# Autodesk Inventor assembly: X-Carriage_LM3011
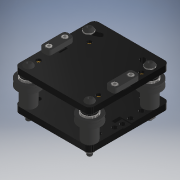
[picture p0: Inventor's stored thumbnail of the model, 180x180]
Saved by Autodesk Inventor 2020.2 (Build 242310000, 310)
## iProperties
Created: 2020-04-03
Part Number: X-Carriage_LM3011
Document SubType Name: Assembly
Designer: rah75
Author: rah75
## Documents named in this file (11)
- C:\Users\rah75\Documents\GitHub\LETU-Maker\CAD\Autodesk Inventor\Base_3001-5999\X-Carriage\Assemblies\X-Carriage_LM3011.iam
- C:\Users\rah75\Documents\GitHub\LETU-Maker\CAD\Autodesk Inventor\Base_3001-5999\X-Carriage\Fabricated_Parts\X-Carraige_Plate_LM3010.ipt
- C:\Users\rah75\Documents\GitHub\LETU-Maker\CAD\Autodesk Inventor\Base_3001-5999\X-Carriage\Printed_Parts\X-Carraige_Spacer_Long_LM3008.ipt
- C:\Users\rah75\Documents\GitHub\LETU-Maker\CAD\Autodesk Inventor\Base_3001-5999\X-Carriage\Printed_Parts\X-Carraige_Spacer_Short_LM3009.ipt
- C:\Users\rah75\Documents\GitHub\LETU-Maker\CAD\Autodesk Inventor\Base_3001-5999\X-Carriage\Printed_Parts\X-Carriage_Belt_Clamp_LM3007.ipt
- C:\Users\rah75\Documents\GitHub\LETU-Maker\CAD\Autodesk Inventor\Stock_Components_1001-2999\Power_Transmission\Bearings\V-Groove_Bearing_5mm_LM1041.ipt
- C:\Users\rah75\Documents\GitHub\LETU-Maker\CAD\Autodesk Inventor\Stock_Components_1001-2999\Fasteners\Nuts\heat_insert_m3_LM1017.ipt
- C:\Users\rah75\Documents\GitHub\LETU-Maker\CAD\Autodesk Inventor\Stock_Components_1001-2999\Fasteners\Screws\SHCS_m3x8_LM1008.ipt
- C:\Users\rah75\Documents\GitHub\LETU-Maker\CAD\Autodesk Inventor\Stock_Components_1001-2999\Fasteners\Washers_Spacers\washer_m5_LM1002.ipt
- C:\Users\rah75\Documents\GitHub\LETU-Maker\CAD\Autodesk Inventor\Stock_Components_1001-2999\Fasteners\Screws\BHHS_m5x50_LM1006.ipt
- C:\Users\rah75\Documents\GitHub\LETU-Maker\CAD\Autodesk Inventor\Stock_Components_1001-2999\Fasteners\Nuts\hex_nut_m5_LM1020.ipt
## Components (40 placed, 10 different names)
1. X-Carraige_Plate_LM3010:1 — Insert:8, Insert:9, Insert:10, Insert:11, Insert:14, Insert:15, Mate:1, Mate:2, Insert:16, Insert:17, Insert:18, Insert:19, Insert:20, Insert:21, Insert:22, Insert:23, Insert:30, Insert:31
2. X-Carraige_Plate_LM3010:2 — Insert:13, Insert:34, Insert:35, Insert:37, Insert:38
3. X-Carraige_Spacer_Long_LM3008:1 — Insert:12
4. X-Carraige_Spacer_Short_LM3009:1 — Insert:4, Insert:9
5. X-Carraige_Spacer_Long_LM3008:2 — Insert:7
6. X-Carraige_Spacer_Short_LM3009:2 — Insert:3, Insert:8
7. X-Carraige_Spacer_Long_LM3008:3 — Insert:5, Insert:13
8. X-Carraige_Spacer_Short_LM3009:3 — Insert:2, Insert:11
9. X-Carraige_Spacer_Long_LM3008:4 — Insert:6
10. X-Carraige_Spacer_Short_LM3009:4 — Insert:1, Insert:10
11. X-Carriage_Belt_Clamp_LM3007:1 — Insert:15, Mate:2, Insert:26, Insert:27
12. X-Carriage_Belt_Clamp_LM3007:2 — Insert:14, Mate:1, Insert:24, Insert:25
13. V-Groove_Bearing_5mm_LM1041:1 — Insert:4, Insert:7
14. V-Groove_Bearing_5mm_LM1041:2 — Insert:3, Insert:5
15. V-Groove_Bearing_5mm_LM1041:3 — Insert:2, Insert:12
16. V-Groove_Bearing_5mm_LM1041:4 — Insert:1, Insert:6
17. heat_insert_m3_LM1017:1 — Insert:18
18. heat_insert_m3_LM1017:2 — Insert:20
19. heat_insert_m3_LM1017:3 — Insert:17
20. heat_insert_m3_LM1017:4 — Insert:16
21. heat_insert_m3_LM1017:5 — Insert:22
22. heat_insert_m3_LM1017:6 — Insert:21
23. heat_insert_m3_LM1017:7 — Insert:23
24. heat_insert_m3_LM1017:8 — Insert:19
25. SHCS_m3x8_LM1008:1 — Insert:24
26. SHCS_m3x8_LM1008:2 — Insert:26
27. SHCS_m3x8_LM1008:3 — Insert:27
28. SHCS_m3x8_LM1008:4 — Insert:25
29. BHHS_m5x50_LM1006:1
30. BHHS_m5x50_LM1006:2
31. BHHS_m5x50_LM1006:3
32. BHHS_m5x50_LM1006:4
33. washer_m5_LM1002:1 — Insert:35, Insert:39
34. washer_m5_LM1002:2 — Insert:34, Insert:36
35. washer_m5_LM1002:3 — Insert:31
36. washer_m5_LM1002:4 — Insert:30
37. hex_nut_m5_LM1020:1 — Insert:39
38. hex_nut_m5_LM1020:2 — Insert:38
39. hex_nut_m5_LM1020:3 — Insert:37
40. hex_nut_m5_LM1020:4 — Insert:36
## Relationships (41: Insert 39, Mate 2)
- Insert:1: X-Carraige_Spacer_Short_LM3009:4 ↔ V-Groove_Bearing_5mm_LM1041:4
- Insert:2: X-Carraige_Spacer_Short_LM3009:3 ↔ V-Groove_Bearing_5mm_LM1041:3
- Insert:3: X-Carraige_Spacer_Short_LM3009:2 ↔ V-Groove_Bearing_5mm_LM1041:2
- Insert:4: X-Carraige_Spacer_Short_LM3009:1 ↔ V-Groove_Bearing_5mm_LM1041:1
- Insert:5: X-Carraige_Spacer_Long_LM3008:3 ↔ V-Groove_Bearing_5mm_LM1041:2
- Insert:6: X-Carraige_Spacer_Long_LM3008:4 ↔ V-Groove_Bearing_5mm_LM1041:4
- Insert:7: X-Carraige_Spacer_Long_LM3008:2 ↔ V-Groove_Bearing_5mm_LM1041:1
- Insert:8: X-Carraige_Plate_LM3010:1 ↔ X-Carraige_Spacer_Short_LM3009:2
- Insert:9: X-Carraige_Plate_LM3010:1 ↔ X-Carraige_Spacer_Short_LM3009:1
- Insert:10: X-Carraige_Plate_LM3010:1 ↔ X-Carraige_Spacer_Short_LM3009:4
- Insert:11: X-Carraige_Plate_LM3010:1 ↔ X-Carraige_Spacer_Short_LM3009:3
- Insert:12: X-Carraige_Spacer_Long_LM3008:1 ↔ V-Groove_Bearing_5mm_LM1041:3
- Insert:13: X-Carraige_Plate_LM3010:2 ↔ X-Carraige_Spacer_Long_LM3008:3
- Insert:14: X-Carraige_Plate_LM3010:1 ↔ X-Carriage_Belt_Clamp_LM3007:2
- Insert:15: X-Carraige_Plate_LM3010:1 ↔ X-Carriage_Belt_Clamp_LM3007:1
- Mate:1: X-Carraige_Plate_LM3010:1 ↔ X-Carriage_Belt_Clamp_LM3007:2
- Mate:2: X-Carraige_Plate_LM3010:1 ↔ X-Carriage_Belt_Clamp_LM3007:1
- Insert:16: X-Carraige_Plate_LM3010:1 ↔ heat_insert_m3_LM1017:4
- Insert:17: X-Carraige_Plate_LM3010:1 ↔ heat_insert_m3_LM1017:3
- Insert:18: X-Carraige_Plate_LM3010:1 ↔ heat_insert_m3_LM1017:1
- Insert:19: X-Carraige_Plate_LM3010:1 ↔ heat_insert_m3_LM1017:8
- Insert:20: X-Carraige_Plate_LM3010:1 ↔ heat_insert_m3_LM1017:2
- Insert:21: X-Carraige_Plate_LM3010:1 ↔ heat_insert_m3_LM1017:6
- Insert:22: X-Carraige_Plate_LM3010:1 ↔ heat_insert_m3_LM1017:5
- Insert:23: X-Carraige_Plate_LM3010:1 ↔ heat_insert_m3_LM1017:7
- Insert:24: X-Carriage_Belt_Clamp_LM3007:2 ↔ SHCS_m3x8_LM1008:1
- Insert:25: X-Carriage_Belt_Clamp_LM3007:2 ↔ SHCS_m3x8_LM1008:4
- Insert:26: X-Carriage_Belt_Clamp_LM3007:1 ↔ SHCS_m3x8_LM1008:2
- Insert:27: X-Carriage_Belt_Clamp_LM3007:1 ↔ SHCS_m3x8_LM1008:3
- [Insert]: BHHS_m5x50_LM1006:4 ↔ washer_m5_LM1002:3
- [Insert]: BHHS_m5x50_LM1006:3 ↔ washer_m5_LM1002:4
- Insert:30: X-Carraige_Plate_LM3010:1 ↔ washer_m5_LM1002:4
- Insert:31: X-Carraige_Plate_LM3010:1 ↔ washer_m5_LM1002:3
- [Insert]: X-Carraige_Plate_LM3010:1 ↔ BHHS_m5x50_LM1006:1
- [Insert]: X-Carraige_Plate_LM3010:1 ↔ BHHS_m5x50_LM1006:2
- Insert:34: X-Carraige_Plate_LM3010:2 ↔ washer_m5_LM1002:2
- Insert:35: X-Carraige_Plate_LM3010:2 ↔ washer_m5_LM1002:1
- Insert:36: washer_m5_LM1002:2 ↔ hex_nut_m5_LM1020:4
- Insert:37: X-Carraige_Plate_LM3010:2 ↔ hex_nut_m5_LM1020:3
- Insert:38: X-Carraige_Plate_LM3010:2 ↔ hex_nut_m5_LM1020:2
- Insert:39: washer_m5_LM1002:1 ↔ hex_nut_m5_LM1020:1
